# Autodesk Inventor assembly: Disk
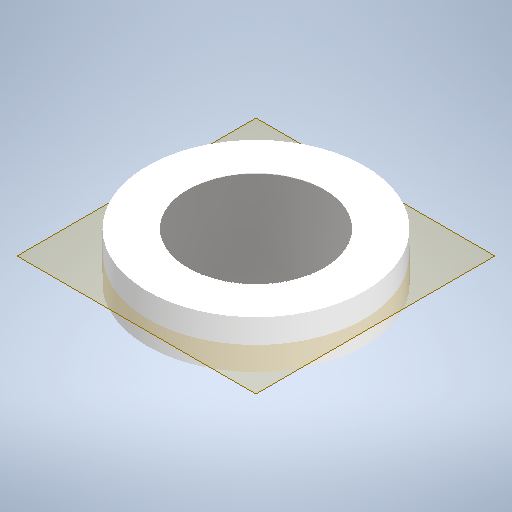
[picture p0: Inventor's stored thumbnail of the model, 512x512]
Saved by Autodesk Inventor 2025.1 (Build 291241020, 241B)
## iProperties
Created: 2024-11-14
Part Number: Disk
Document SubType Name: Assembly
Designer: leon-
Author: leon-
## Documents named in this file (3)
- C:\Users\leon-\OneDrive\Dokumente\Education\Berkeley\Embedded_Systems\Project\CAD_Model\Disk.iam
- C:\Users\leon-\OneDrive\Dokumente\Education\Berkeley\Embedded_Systems\Project\CAD_Model\3DPrint_Parts\Disk.ipt
- C:\Users\leon-\OneDrive\Dokumente\Education\Berkeley\Embedded_Systems\Project\CAD_Model\Purchase_Parts\Mechanical\Steel_Inserts.ipt
## Components (2 placed, 2 different names)
1. Disk:1 — Mate:1, Mate:2
2. Steel_Inserts:1 — Mate:1, Mate:2
## Relationships (2: Mate 2)
- Mate:1: Disk:1 ↔ Steel_Inserts:1
- Mate:2: Disk:1 ↔ Steel_Inserts:1
